# Autodesk Inventor assembly: base_MIR
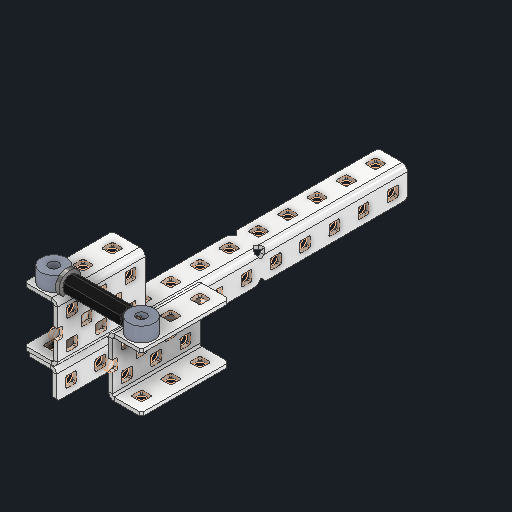
[picture p0: Inventor's stored thumbnail of the model, 512x512]
Saved by Autodesk Inventor 2024 (Build 280153000, 153)
## iProperties
Created: 2023-10-22
Part Number: base_MIR
Document SubType Name: Assembly
Designer: Averey Ku
Author: Averey Ku
## Documents named in this file (8)
- D:\vex_robotics\hardware\cad\spades_v0.1\intake\mirrored_parts\base_MIR.iam
- D:\vex_robotics\hardware\cad\spades_v0.1\intake\mirrored_parts\Alu C 1x2x1x3_MIR.ipt
- D:\vex_robotics\hardware\cad\spades_v0.1\intake\mirrored_parts\Shaft Collar No Screw_MIR.ipt
- D:\vex_robotics\hardware\cad\VEX-CAD-Inventor-1.41\Structure\Standoff\Standoff 1.00.ipt
- D:\vex_robotics\hardware\cad\VEX-CAD-Inventor-1.41\Structure\Standoff.ipt
- D:\vex_robotics\hardware\cad\VEX-CAD-Inventor-1.41\Motion\Spacers\Washer Steel\SWasher .375 OD x .062500.ipt
- D:\vex_robotics\hardware\cad\VEX-CAD-Inventor-1.41\Motion\Spacers\Washer Steel.ipt
- D:\vex_robotics\hardware\cad\spades_v0.1\intake\mirrored_parts\Alu Angle 1x1x12_MIR.ipt
## Components (7 placed, 5 different names)
1. Alu C 1x2x1x3_MIR:1 — Mate:1, Insert:1, Insert:2, Mate:3, Insert:6
2. Alu C 1x2x1x3_MIR:2 — Mate:1, Insert:1, Insert:3
3. Shaft Collar No Screw_MIR:1 — Insert:2, Mate:2, Angle:1, Insert:5
4. Shaft Collar No Screw_MIR:2 — Mate:2, Angle:1, Insert:3
5. Standoff 1.00:1 — Insert:4
6. SWasher .375 OD x .062500:1 — Insert:5, Insert:4
7. Alu Angle 1x1x12_MIR:1 — Mate:3, Insert:6
## Relationships (10: Insert 6, Mate 3, Angle 1)
- Mate:1: Alu C 1x2x1x3_MIR:1 ↔ Alu C 1x2x1x3_MIR:2
- Insert:1 (22.225 mm): Alu C 1x2x1x3_MIR:1 ↔ Alu C 1x2x1x3_MIR:2
- Insert:2: Alu C 1x2x1x3_MIR:1 ↔ Shaft Collar No Screw_MIR:1
- Mate:2: Shaft Collar No Screw_MIR:1 ↔ Shaft Collar No Screw_MIR:2
- Angle:1 (0 deg): Shaft Collar No Screw_MIR:1 ↔ Shaft Collar No Screw_MIR:2
- Insert:3: Alu C 1x2x1x3_MIR:2 ↔ Shaft Collar No Screw_MIR:2
- Insert:5: Shaft Collar No Screw_MIR:1 ↔ SWasher .375 OD x .062500:1
- Insert:4: Standoff 1.00:1 ↔ SWasher .375 OD x .062500:1
- Mate:3: Alu C 1x2x1x3_MIR:1 ↔ Alu Angle 1x1x12_MIR:1
- Insert:6: Alu C 1x2x1x3_MIR:1 ↔ Alu Angle 1x1x12_MIR:1
